# Autodesk Inventor assembly: LandingSystem on LandingBase
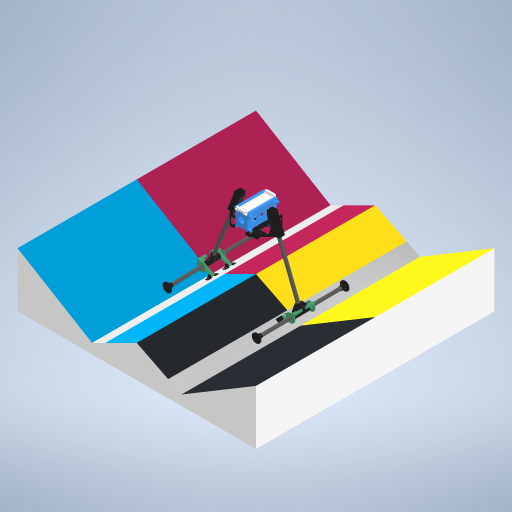
[picture p0: Inventor's stored thumbnail of the model, 512x512]
Saved by Autodesk Inventor 2023 (Build 270158000, 158)
## iProperties
Created: 2023-04-23
Part Number: LandingSystem on LandingBase
Document SubType Name: Assembly
Designer: ethan
Author: ethan
## Documents named in this file (3)
- D:\Documents\GitHub\WU-Team20-AutonomousDrone\CAD\ASSEMBLY\LandingSystem on LandingBase.iam
- D:\Documents\GitHub\WU-Team20-AutonomousDrone\CAD\Charging Base\Drone Charging Base.ipt
- D:\Documents\GitHub\WU-Team20-AutonomousDrone\CAD\ASSEMBLY\SubAssembly - EntireLandingSystem.iam
## Components (2 placed, 2 different names)
1. Drone Charging Base:1 — Flush:1, Flush:2, Flush:3
2. SubAssembly - EntireLandingSystem:1 [sub-assembly] — Flush:1, Flush:2, Flush:3
## Relationships (3: Flush 3)
- Flush:1 (579.6 mm): Drone Charging Base:1 ↔ SubAssembly - EntireLandingSystem:1
- Flush:2 (534.6 mm): Drone Charging Base:1 ↔ SubAssembly - EntireLandingSystem:1
- Flush:3 (406.4 mm): Drone Charging Base:1 ↔ SubAssembly - EntireLandingSystem:1
